# Autodesk Inventor assembly: HitBox
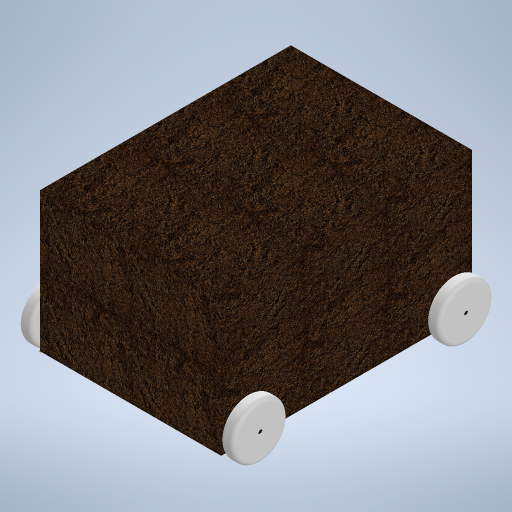
[picture p0: Inventor's stored thumbnail of the model, 512x512]
Saved by Autodesk Inventor 2023 (Build 270158000, 158)
## iProperties
Created: 2022-09-21
Part Number: HitBox
Document SubType Name: Assembly
Designer: PC
Mass: 312557 g
Surface Area: 31626.2 cm^2
Volume: 312557 cm^3
Density: 1 g/cm^3
Author: PC
## Documents named in this file (3)
- C:\Users\PC\Documents\PersonalCAD\ARCIGVC\IGVC-Robot\GazeboR1\FullAttempt\HitBox\HitBox.iam
- C:\Users\PC\Documents\PersonalCAD\ARCIGVC\IGVC-Robot\GazeboR1\FullAttempt\HitBox\Frame.ipt
- C:\Users\PC\Documents\PersonalCAD\ARCIGVC\IGVC-Robot\GazeboR1\FullAttempt\HitBox\Wheel.ipt
## Components (5 placed, 2 different names)
1. Frame:1 — Mate:1, Flush:1, Mate:2, Flush:2, Mate:3, Flush:3, Mate:4, Flush:4, Mate:5, Flush:5, Mate:6
2. Wheel:1 — Mate:1, Flush:1
3. Wheel:2 — Mate:4, Flush:4
4. Wheel:3 — Mate:2, Flush:2
5. Wheel:4 — Mate:3, Flush:3
## Relationships (11: Mate 6, Flush 5)
- Mate:1: Frame:1 ↔ Wheel:1
- Flush:1 (61.5442 mm): Frame:1 ↔ Wheel:1
- Mate:2: Frame:1 ↔ Wheel:3
- Flush:2 (-61.5442 mm): Frame:1 ↔ Wheel:3
- Mate:3: Frame:1 ↔ Wheel:4
- Flush:3 (61.5442 mm): Frame:1 ↔ Wheel:4
- Mate:4: Frame:1 ↔ Wheel:2
- Flush:4 (61.5442 mm): Frame:1 ↔ Wheel:2
- Mate:5: Frame:1
- Flush:5: Frame:1
- Mate:6: Frame:1
